# Autodesk Inventor assembly: 6P Sprocket
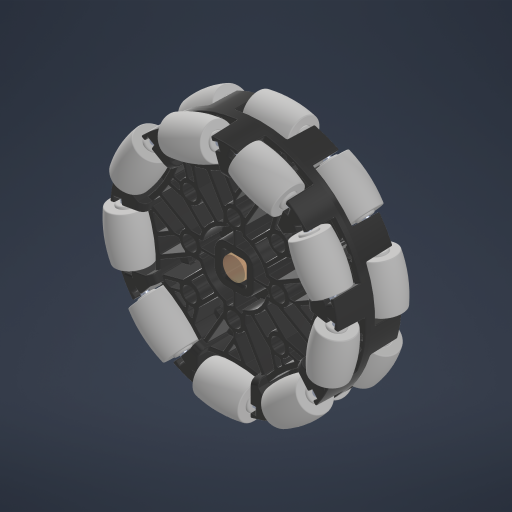
[picture p0: Inventor's stored thumbnail of the model, 512x512]
Saved by Autodesk Inventor 2023.2 (Build 272271000, 271)
## iProperties
Created: 2022-08-02
Part Number: 6P Sprocket
Document SubType Name: Assembly
Designer: ylu12
Author: ylu12
## Documents named in this file (3)
- D:\CAD\Parts\standard\Motion\Wheels\Omni Wheels\Omni Wheel\2.75 Omni AS, No Insert.iam
- D:\CAD\Parts\standard\Motion\Wheels\Omni Wheels\Reference Parts\2.75 Omni Antistatic.ipt
- D:\CAD\Parts\standard\Motion\Wheels\Omni Wheels\Omni Wheel.iam
## Components (1 placed, 1 different names)
1. 2.75 Omni Antistatic
## Relationships (3: Mate 2, Flush 1)
- [Flush]: 2.75 Omni Antistatic
- [Mate]: 2.75 Omni Antistatic
- [Mate]: 2.75 Omni Antistatic
